# Autodesk Inventor assembly: WheelAssemble2.0 - left1
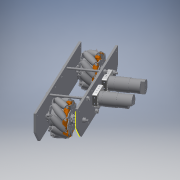
[picture p0: Inventor's stored thumbnail of the model, 180x180]
Saved by Autodesk Inventor 2017 (Build 210142000, 142)
## iProperties
Created: 2016-09-10
Part Number: WheelAssemble2.0 - left1
Document SubType Name: Assembly
Designer: RoboticsUser
Author: RoboticsUser
## Documents named in this file (14)
- C:\Robotics\CAD\2016-17_CAD\WheelAssemble2.0 - left1.iam
- C:\Robotics\CAD\COTSParts\Actobotics\545 parts\545556.ipt
- C:\Robotics\CAD\COTSParts\Actobotics\615 parts\615102.ipt
- C:\Robotics\CAD\COTSParts\Actobotics\634 parts\634080.ipt
- C:\Robotics\CAD\COTSParts\Motors\Andymark 2964  NeveRest 40 Motor.ipt
- C:\Robotics\CAD\COTSParts\Tetrix\tetrix-motor-mounts-1.snapshot.1\Tetrex 2pc motor mount.ipt
- C:\Robotics\CAD\COTSParts\Actobotics\545 parts\545456.ipt
- C:\Robotics\CAD\COTSParts\Wheels\AndyMark Mecanum Wheels\100mm Aluminum Mecanum wheels.ipt
- C:\Robotics\CAD\2016-17_CAD\DrainTrainPlate2.0.iam
- C:\Robotics\CAD\2016-17_CAD\DriveTrainPlate -Inside.ipt
- C:\Robotics\CAD\COTSParts\Actobotics\535 parts\535198.ipt
- C:\Robotics\CAD\COTSParts\Actobotics\collar.ipt
- C:\Robotics\CAD\2016-17_CAD\13019-Fastenal-07-11-2017.ipt
- C:\Robotics\CAD\2016-17_CAD\1137018-Fastenal-07-11-2017.ipt
## Components (38 placed, 13 different names)
1. 545556:2 — Mate:10, Mate:13, Mate:47
2. 615102:4 — Mate:114
3. 634080:2 — Mate:10, Mate:12, Mate:26, Mate:45, Mate:56, Insert:117, Mate:95, Mate:101
4. 545556:6 — Insert:83, Mate:73
5. 634080:3 — Mate:28, Mate:50, Mate:68, Mate:74, Insert:118, Mate:93, Mate:100
6. Andymark 2964  NeveRest 40 Motor:2 — Mate:118, Mate:119
7. 545556:8 — Insert:121, Mate:119
8. 545556:9 — Mate:113, Mate:114
9. Andymark 2964  NeveRest 40 Motor:3 — Mate:112, Mate:113, Flush:2
10. Tetrex 2pc motor mount:2 — Mate:110, Mate:111, Mate:112
11. 545456:1 — Mate:12, Mate:13, Insert:89
12. 545456:3 — Insert:83, Insert:88
13. 615102:6 — Insert:121, Mate:104
14. 615102:7 — Mate:45, Mate:47, Mate:70
15. 100mm Aluminum Mecanum wheels:1 — Insert:88, Mate:27, Mate:50
16. 100mm Aluminum Mecanum wheels:2 — Insert:89, Mate:25
17. 545456:4 — Mate:25, Mate:26, Insert:116
18. 545456:5 — Mate:27, Mate:28, Insert:115
19. 545556:12 — Insert:115, Mate:106
20. 545556:13 — Insert:116
21. DrainTrainPlate2.0:1 [sub-assembly] — Mate:56, Mate:68, Mate:85, Mate:86, Mate:97, Mate:98, Mate:106, Mate:107, Mate:108, Mate:120, Mate:121, Mate:122, Mate:123, Mate:124, Mate:125
22. DriveTrainPlate -Inside:1 — Mate:70, Mate:83, Mate:87, Mate:88, Mate:96, Mate:104, Mate:105, Mate:110, Mate:111, Flush:2, Mate:115, Mate:116, Mate:117, Mate:126, Mate:127, Mate:128
23. 615102:8 — Mate:73, Mate:74, Mate:83
24. 535198:2 — Mate:85, Mate:97
25. 535198:3 — Mate:88, Mate:100
26. 535198:4 — Mate:87, Mate:101
27. 535198:5 — Mate:86, Mate:98
28. collar:1 — Insert:117, Mate:107
29. collar:2 — Insert:118, Mate:108
30. Tetrex 2pc motor mount:3 — Mate:115, Mate:116, Mate:117, Mate:118
31. collar:3 — Mate:95, Mate:96
32. collar:4 — Mate:93, Mate:105
33. 13019-Fastenal-07-11-2017:1 — Mate:123, Mate:125, Mate:129
34. 13019-Fastenal-07-11-2017:2 — Mate:120, Mate:121
35. 13019-Fastenal-07-11-2017:3 — Mate:122, Mate:124
36. 1137018-Fastenal-07-11-2017:1 — Mate:129
37. 1137018-Fastenal-07-11-2017:2 — Mate:126
38. 1137018-Fastenal-07-11-2017:3 — Mate:127, Mate:128
## Relationships (61: Mate 52, Insert 8, Flush 1)
- Insert:83: 545556:6 ↔ 545456:3
- Mate:10: 545556:2 ↔ 634080:2
- Mate:12: 634080:2 ↔ 545456:1
- Mate:13: 545556:2 ↔ 545456:1
- Insert:88: 545456:3 ↔ 100mm Aluminum Mecanum wheels:1
- Insert:89: 545456:1 ↔ 100mm Aluminum Mecanum wheels:2
- Mate:25: 100mm Aluminum Mecanum wheels:2 ↔ 545456:4
- Mate:26: 634080:2 ↔ 545456:4
- Mate:27: 100mm Aluminum Mecanum wheels:1 ↔ 545456:5
- Mate:28: 634080:3 ↔ 545456:5
- Mate:45: 634080:2 ↔ 615102:7
- Mate:47: 545556:2 ↔ 615102:7
- Mate:50: 634080:3 ↔ 100mm Aluminum Mecanum wheels:1
- Mate:56: 634080:2 ↔ DrainTrainPlate2.0:1
- Mate:68: 634080:3 ↔ DrainTrainPlate2.0:1
- Mate:70 (6.35 mm): 615102:7 ↔ DriveTrainPlate -Inside:1
- Mate:73: 545556:6 ↔ 615102:8
- Mate:74: 634080:3 ↔ 615102:8
- Insert:115: 545456:5 ↔ 545556:12
- Mate:83 (6.35 mm): DriveTrainPlate -Inside:1 ↔ 615102:8
- Insert:116: 545456:4 ↔ 545556:13
- Mate:85: DrainTrainPlate2.0:1 ↔ 535198:2
- Mate:86: DrainTrainPlate2.0:1 ↔ 535198:5
- Mate:87: DriveTrainPlate -Inside:1 ↔ 535198:4
- Mate:88: DriveTrainPlate -Inside:1 ↔ 535198:3
- Insert:117: 634080:2 ↔ collar:1
- Insert:118 (-6.35 mm): 634080:3 ↔ collar:2
- Mate:93: 634080:3 ↔ collar:4
- Mate:95: 634080:2 ↔ collar:3
- Mate:96: DriveTrainPlate -Inside:1 ↔ collar:3
- Mate:97: DrainTrainPlate2.0:1 ↔ 535198:2
- Mate:98: DrainTrainPlate2.0:1 ↔ 535198:5
- Mate:100: 634080:3 ↔ 535198:3
- Mate:101: 634080:2 ↔ 535198:4
- Insert:121: 545556:8 ↔ 615102:6
- Mate:104 (3.175 mm): 615102:6 ↔ DriveTrainPlate -Inside:1
- Mate:105: DriveTrainPlate -Inside:1 ↔ collar:4
- Mate:106 (3.175 mm): 545556:12 ↔ DrainTrainPlate2.0:1
- Mate:107: DrainTrainPlate2.0:1 ↔ collar:1
- Mate:108: DrainTrainPlate2.0:1 ↔ collar:2
- Mate:110: Tetrex 2pc motor mount:2 ↔ DriveTrainPlate -Inside:1
- Mate:111: Tetrex 2pc motor mount:2 ↔ DriveTrainPlate -Inside:1
- Mate:112: Andymark 2964  NeveRest 40 Motor:3 ↔ Tetrex 2pc motor mount:2
- Mate:113: 545556:9 ↔ Andymark 2964  NeveRest 40 Motor:3
- Flush:2: Andymark 2964  NeveRest 40 Motor:3 ↔ DriveTrainPlate -Inside:1
- Mate:114: 615102:4 ↔ 545556:9
- Mate:115: DriveTrainPlate -Inside:1 ↔ Tetrex 2pc motor mount:3
- Mate:116: DriveTrainPlate -Inside:1 ↔ Tetrex 2pc motor mount:3
- Mate:117: DriveTrainPlate -Inside:1 ↔ Tetrex 2pc motor mount:3
- Mate:118: Andymark 2964  NeveRest 40 Motor:2 ↔ Tetrex 2pc motor mount:3
- Mate:119: Andymark 2964  NeveRest 40 Motor:2 ↔ 545556:8
- Mate:120: DrainTrainPlate2.0:1 ↔ 13019-Fastenal-07-11-2017:2
- Mate:121: DrainTrainPlate2.0:1 ↔ 13019-Fastenal-07-11-2017:2
- Mate:122: DrainTrainPlate2.0:1 ↔ 13019-Fastenal-07-11-2017:3
- Mate:123: DrainTrainPlate2.0:1 ↔ 13019-Fastenal-07-11-2017:1
- Mate:124: DrainTrainPlate2.0:1 ↔ 13019-Fastenal-07-11-2017:3
- Mate:125: DrainTrainPlate2.0:1 ↔ 13019-Fastenal-07-11-2017:1
- Mate:126: DriveTrainPlate -Inside:1 ↔ 1137018-Fastenal-07-11-2017:2
- Mate:127: DriveTrainPlate -Inside:1 ↔ 1137018-Fastenal-07-11-2017:3
- Mate:128: DriveTrainPlate -Inside:1 ↔ 1137018-Fastenal-07-11-2017:3
- Mate:129: 13019-Fastenal-07-11-2017:1 ↔ 1137018-Fastenal-07-11-2017:1
